# Autodesk Inventor assembly: Robot
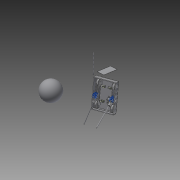
[picture p0: Inventor's stored thumbnail of the model, 180x180]
Saved by Autodesk Inventor 2014 (Build 180170000, 170)
## iProperties
Created: 2014-01-21
Part Number: Robot
Document SubType Name: Assembly
Designer: NilesStanton
Author: NilesStanton
## Documents named in this file (23)
- C:\GitHub\team3566-2014\CAD\Robot.iam
- C:\FIRST-2014-KOP\Additions\2014 Sidings.ipt
- C:\FIRST-2014-KOP\Motors\MOT_CIM-Motor_217-2000.iam
- C:\FIRST-2014-KOP\Additions\Flat Board.ipt
- C:\FIRST-2014-KOP\Additions\Front Paneling.ipt
- C:\FIRST-2014-KOP\Additions\3.5 in spacer.ipt
- C:\FIRST-2014-KOP\Additions\Mechanum Wheel.ipt
- C:\FIRST-2014-KOP\Additions\Gearbox.ipt
- C:\FIRST-2014-KOP\Additions\Long Bumber Wood.ipt
- C:\FIRST-2014-KOP\Additions\Short Bumper Wood.ipt
- C:\FIRST-2014-KOP\Drive Base Kit\DBK_TBMiniHousing-am-0650.ipt
- C:\FIRST-2014-KOP\Additions\El Tauro Horns.ipt
- C:\FIRST-2014-KOP\Additions\Tauro Vertical Pivot.ipt
- C:\FIRST-2014-KOP\Additions\Tauro Spacer.ipt
- C:\FIRST-2014-KOP\Additions\Tauro Vertical Pivot part 2.ipt
- C:\FIRST-2014-KOP\Additions\3.5 in pole.ipt
- C:\FIRST-2014-KOP\Additions\motor casing.ipt
- C:\FIRST-2014-KOP\Additions\.5 in spacer ring.ipt
- C:\FIRST-2014-KOP\Additions\winch triangle.ipt
- C:\FIRST-2014-KOP\Additions\Winch.ipt
- C:\FIRST-2014-KOP\Motors\MOT_GearMotor_am-0914.ipt
- C:\FIRST-2014-KOP\Additions\Bottom Board.ipt
- C:\GitHub\team3566-2014\CAD\ball.ipt
## Components (51 placed, 22 different names)
1. 2014 Sidings:1 — Flush:8, Mate:4, Angle:5, Flush:19, Flush:37, Flush:38, Flush:49, Mate:18
2. 2014 Sidings:2 — Mate:3, Flush:3, Angle:3, Flush:11, Flush:14, Flush:15, Tangent:7, Tangent:8, Flush:22, Flush:23, Flush:25, Flush:26, Flush:30, Flush:31, Mate:16
3. MOT_CIM-Motor_217-2000:1 [sub-assembly] — Tangent:9, Flush:30, Tangent:10
4. MOT_CIM-Motor_217-2000:2 [sub-assembly] — Flush:31, Tangent:11, Tangent:12
5. MOT_CIM-Motor_217-2000:3 [sub-assembly] — Flush:33, Tangent:15, Tangent:16
6. MOT_CIM-Motor_217-2000:4 [sub-assembly] — Flush:32, Tangent:13, Tangent:14
7. Flat Board:1
8. 2014 Sidings:3
9. Front Paneling:1 — Mate:2, Flush:2, Angle:2, Mate:3, Flush:3, Angle:3, Flush:24, Flush:27, Tangent:9, Tangent:15, Mate:7, Flush:55
10. Front Paneling:2 — Mate:1, Flush:1, Angle:1, Flush:5, Flush:7, Flush:9, Flush:10, Flush:18, Flush:21, Tangent:12, Tangent:13, Flush:36, Flush:39, Mate:6
11. 3.5 in spacer:1 — Flush:9, Flush:10, Flush:11, Flush:12, Flush:13, Mate:5, Angle:6, Tangent:1, Tangent:2
12. 3.5 in spacer:2 — Flush:5, Flush:6, Angle:4, Flush:7, Flush:8, Mate:4, Angle:5, Tangent:3, Tangent:4
13. 2014 Sidings:4 — Flush:12, Flush:13, Mate:5, Angle:6, Flush:34, Flush:35, Flush:52
14. 2014 Sidings:5 — Mate:1, Flush:1, Angle:1, Mate:2, Flush:2, Angle:2, Flush:6, Angle:4, Flush:16, Flush:17, Tangent:5, Tangent:6, Flush:20, Flush:28, Flush:29, Flush:32, Flush:33
15. Mechanum Wheel:1 — Flush:14, Tangent:1, Tangent:7
16. Mechanum Wheel:2 — Flush:17, Tangent:4, Tangent:5
17. Mechanum Wheel:3 — Flush:15, Tangent:2, Tangent:8
18. Mechanum Wheel:4 — Flush:16, Tangent:3, Tangent:6
19. Gearbox:1 — Flush:27, Flush:28, Flush:29, Tangent:16
20. Gearbox:2 — Flush:24, Flush:25, Flush:26, Tangent:10
21. Gearbox:3 — Flush:18, Flush:19, Flush:20, Tangent:14
22. Gearbox:4 — Flush:21, Flush:22, Flush:23, Tangent:11
23. Long Bumber Wood:1 — Flush:34, Flush:35, Flush:36, Flush:43, Flush:44, Flush:53
24. Long Bumber Wood:2 — Flush:37, Flush:38, Flush:39, Flush:41, Flush:42, Flush:50
25. Short Bumper Wood:1 — Flush:41, Mate:6, Flush:42, Tangent:21, Tangent:22
26. Short Bumper Wood:2 — Mate:7, Flush:43, Flush:44
27. DBK_TBMiniHousing-am-0650:1 — Insert:1, Flush:45, Flush:52, Flush:53
28. DBK_TBMiniHousing-am-0650:2 — Insert:2, Flush:45
29. El Tauro Horns:1
30. El Tauro Horns:2 — Mate:11, Insert:7
31. Tauro Vertical Pivot:1 — Insert:1, Insert:2, Insert:3, Tangent:22
32. Tauro Spacer:1 — Mate:8, Mate:9, Flush:46, Insert:3
33. Tauro Vertical Pivot part 2:1 — Mate:8, Mate:9, Flush:46, Insert:4, Insert:5
34. 3.5 in pole:1 — Insert:4, Insert:5, Insert:6
35. motor casing:1 — Insert:6, Mate:10, Tangent:17, Tangent:18
36. .5 in spacer ring:1 — Mate:10, Tangent:17, Tangent:18, Mate:11, Insert:7
37. DBK_TBMiniHousing-am-0650:3
38. DBK_TBMiniHousing-am-0650:4 — Flush:49, Flush:50
39. El Tauro Horns:3
40. Tauro Vertical Pivot:2 — Tangent:21
41. Tauro Spacer:2
42. Tauro Vertical Pivot part 2:2
43. 3.5 in pole:2
44. motor casing:2
45. .5 in spacer ring:2
46. winch triangle:1 — Insert:16, Flush:54
47. winch triangle:2 — Insert:15, Flush:54, Mate:17
48. Winch:1 — Insert:15, Insert:16, Insert:17
49. MOT_GearMotor_am-0914:1 — Insert:17, Mate:18
50. Bottom Board:1 — Mate:16, Flush:55, Mate:17
51. ball:1
## Relationships (115: Flush 52, Tangent 22, Mate 18, Insert 17, Angle 6)
- Mate:1: Front Paneling:2 ↔ 2014 Sidings:5
- Flush:1: Front Paneling:2 ↔ 2014 Sidings:5
- Angle:1 (90 deg): Front Paneling:2 ↔ 2014 Sidings:5
- Mate:2: Front Paneling:1 ↔ 2014 Sidings:5
- Flush:2: Front Paneling:1 ↔ 2014 Sidings:5
- Angle:2 (90 deg): Front Paneling:1 ↔ 2014 Sidings:5
- Mate:3: 2014 Sidings:2 ↔ Front Paneling:1
- Flush:3: 2014 Sidings:2 ↔ Front Paneling:1
- Angle:3 (90 deg): 2014 Sidings:2 ↔ Front Paneling:1
- Flush:5: Front Paneling:2 ↔ 3.5 in spacer:2
- Flush:6: 3.5 in spacer:2 ↔ 2014 Sidings:5
- Angle:4 (90 deg): 3.5 in spacer:2 ↔ 2014 Sidings:5
- Flush:7: Front Paneling:2 ↔ 3.5 in spacer:2
- Flush:8: 2014 Sidings:1 ↔ 3.5 in spacer:2
- Mate:4: 2014 Sidings:1 ↔ 3.5 in spacer:2
- Angle:5 (90 deg): 2014 Sidings:1 ↔ 3.5 in spacer:2
- Flush:9: Front Paneling:2 ↔ 3.5 in spacer:1
- Flush:10: Front Paneling:2 ↔ 3.5 in spacer:1
- Flush:11: 2014 Sidings:2 ↔ 3.5 in spacer:1
- Flush:12: 3.5 in spacer:1 ↔ 2014 Sidings:4
- Flush:13: 3.5 in spacer:1 ↔ 2014 Sidings:4
- Mate:5: 3.5 in spacer:1 ↔ 2014 Sidings:4
- Angle:6 (90 deg): 3.5 in spacer:1 ↔ 2014 Sidings:4
- Flush:14: 2014 Sidings:2 ↔ Mechanum Wheel:1
- Flush:15: 2014 Sidings:2 ↔ Mechanum Wheel:3
- Tangent:1 (50.8 mm): 3.5 in spacer:1 ↔ Mechanum Wheel:1
- Tangent:2 (622.3 mm): 3.5 in spacer:1 ↔ Mechanum Wheel:3
- Flush:16: 2014 Sidings:5 ↔ Mechanum Wheel:4
- Flush:17: 2014 Sidings:5 ↔ Mechanum Wheel:2
- Tangent:3 (50.8 mm): 3.5 in spacer:2 ↔ Mechanum Wheel:4
- Tangent:4 (622.3 mm): 3.5 in spacer:2 ↔ Mechanum Wheel:2
- Tangent:5 (-38.1 mm): 2014 Sidings:5 ↔ Mechanum Wheel:2
- Tangent:6 (-38.1 mm): 2014 Sidings:5 ↔ Mechanum Wheel:4
- Tangent:7 (-38.1 mm): 2014 Sidings:2 ↔ Mechanum Wheel:1
- Tangent:8 (-38.1 mm): 2014 Sidings:2 ↔ Mechanum Wheel:3
- Flush:18 (88.9 mm): Front Paneling:2 ↔ Gearbox:3
- Flush:19 (18.796 mm): 2014 Sidings:1 ↔ Gearbox:3
- Flush:20 (6.35 mm): 2014 Sidings:5 ↔ Gearbox:3
- Flush:21 (88.9 mm): Front Paneling:2 ↔ Gearbox:4
- Flush:22 (6.35 mm): 2014 Sidings:2 ↔ Gearbox:4
- Flush:23 (19.05 mm): 2014 Sidings:2 ↔ Gearbox:4
- Flush:24 (88.9 mm): Front Paneling:1 ↔ Gearbox:2
- Flush:25 (6.35 mm): 2014 Sidings:2 ↔ Gearbox:2
- Flush:26 (19.05 mm): 2014 Sidings:2 ↔ Gearbox:2
- Flush:27 (88.9 mm): Front Paneling:1 ↔ Gearbox:1
- Flush:28 (19.05 mm): 2014 Sidings:5 ↔ Gearbox:1
- Flush:29 (6.35 mm): 2014 Sidings:5 ↔ Gearbox:1
- Tangent:9 (215.9 mm): MOT_CIM-Motor_217-2000:1 ↔ Front Paneling:1
- Flush:30 (44.45 mm): 2014 Sidings:2 ↔ MOT_CIM-Motor_217-2000:1
- Tangent:10 (6.35 mm): MOT_CIM-Motor_217-2000:1 ↔ Gearbox:2
- Flush:31 (44.45 mm): 2014 Sidings:2 ↔ MOT_CIM-Motor_217-2000:2
- Tangent:11 (6.35 mm): MOT_CIM-Motor_217-2000:2 ↔ Gearbox:4
- Tangent:12 (215.9 mm): MOT_CIM-Motor_217-2000:2 ↔ Front Paneling:2
- Flush:32 (44.45 mm): MOT_CIM-Motor_217-2000:4 ↔ 2014 Sidings:5
- Tangent:13 (215.9 mm): MOT_CIM-Motor_217-2000:4 ↔ Front Paneling:2
- Tangent:14 (6.35 mm): MOT_CIM-Motor_217-2000:4 ↔ Gearbox:3
- Flush:33 (44.45 mm): MOT_CIM-Motor_217-2000:3 ↔ 2014 Sidings:5
- Tangent:15 (215.9 mm): MOT_CIM-Motor_217-2000:3 ↔ Front Paneling:1
- Tangent:16 (6.35 mm): MOT_CIM-Motor_217-2000:3 ↔ Gearbox:1
- Flush:34 (6.35 mm): 2014 Sidings:4 ↔ Long Bumber Wood:1
- Flush:35 (-76.2 mm): 2014 Sidings:4 ↔ Long Bumber Wood:1
- Flush:36: Front Paneling:2 ↔ Long Bumber Wood:1
- Flush:37 (6.35 mm): 2014 Sidings:1 ↔ Long Bumber Wood:2
- Flush:38 (-76.2 mm): 2014 Sidings:1 ↔ Long Bumber Wood:2
- Flush:39: Front Paneling:2 ↔ Long Bumber Wood:2
- Flush:41: Long Bumber Wood:2 ↔ Short Bumper Wood:1
- Mate:6: Front Paneling:2 ↔ Short Bumper Wood:1
- Flush:42: Long Bumber Wood:2 ↔ Short Bumper Wood:1
- Mate:7: Front Paneling:1 ↔ Short Bumper Wood:2
- Flush:43: Long Bumber Wood:1 ↔ Short Bumper Wood:2
- Flush:44: Long Bumber Wood:1 ↔ Short Bumper Wood:2
- Insert:1 (-50.8 mm): DBK_TBMiniHousing-am-0650:1 ↔ Tauro Vertical Pivot:1
- Insert:2 (-50.8 mm): DBK_TBMiniHousing-am-0650:2 ↔ Tauro Vertical Pivot:1
- Flush:45: DBK_TBMiniHousing-am-0650:1 ↔ DBK_TBMiniHousing-am-0650:2
- Mate:8: Tauro Spacer:1 ↔ Tauro Vertical Pivot part 2:1
- Mate:9 (19.05 mm): Tauro Spacer:1 ↔ Tauro Vertical Pivot part 2:1
- Flush:46 (3.175 mm): Tauro Spacer:1 ↔ Tauro Vertical Pivot part 2:1
- Insert:3 (-76.2 mm): Tauro Vertical Pivot:1 ↔ Tauro Spacer:1
- Insert:4: Tauro Vertical Pivot part 2:1 ↔ 3.5 in pole:1
- Insert:5: Tauro Vertical Pivot part 2:1 ↔ 3.5 in pole:1
- Insert:6 (6.35 mm): 3.5 in pole:1 ↔ motor casing:1
- Mate:10: motor casing:1 ↔ .5 in spacer ring:1
- Tangent:17 (38.1 mm): motor casing:1 ↔ .5 in spacer ring:1
- Tangent:18 (31.75 mm): motor casing:1 ↔ .5 in spacer ring:1
- Mate:11: El Tauro Horns:2 ↔ .5 in spacer ring:1
- Insert:7: El Tauro Horns:2 ↔ .5 in spacer ring:1
- [Insert] (-50.8 mm): DBK_TBMiniHousing-am-0650:3 ↔ Tauro Vertical Pivot:2
- [Insert] (-50.8 mm): DBK_TBMiniHousing-am-0650:4 ↔ Tauro Vertical Pivot:2
- [Flush]: DBK_TBMiniHousing-am-0650:3 ↔ DBK_TBMiniHousing-am-0650:4
- [Mate]: Tauro Spacer:2 ↔ Tauro Vertical Pivot part 2:2
- [Mate] (19.05 mm): Tauro Spacer:2 ↔ Tauro Vertical Pivot part 2:2
- [Flush] (3.175 mm): Tauro Spacer:2 ↔ Tauro Vertical Pivot part 2:2
- [Insert] (-76.2 mm): Tauro Vertical Pivot:2 ↔ Tauro Spacer:2
- [Insert]: Tauro Vertical Pivot part 2:2 ↔ 3.5 in pole:2
- [Insert]: Tauro Vertical Pivot part 2:2 ↔ 3.5 in pole:2
- [Insert] (6.35 mm): 3.5 in pole:2 ↔ motor casing:2
- [Mate]: motor casing:2 ↔ .5 in spacer ring:2
- [Tangent] (38.1 mm): motor casing:2 ↔ .5 in spacer ring:2
- [Tangent] (31.75 mm): motor casing:2 ↔ .5 in spacer ring:2
- [Mate]: El Tauro Horns:3 ↔ .5 in spacer ring:2
- [Insert]: El Tauro Horns:3 ↔ .5 in spacer ring:2
- Flush:49 (-25.4 mm): 2014 Sidings:1 ↔ DBK_TBMiniHousing-am-0650:4
- Flush:50 (45.72 mm): Long Bumber Wood:2 ↔ DBK_TBMiniHousing-am-0650:4
- Tangent:21 (342.9 mm): Short Bumper Wood:1 ↔ Tauro Vertical Pivot:2
- Flush:52 (-25.4 mm): 2014 Sidings:4 ↔ DBK_TBMiniHousing-am-0650:1
- Flush:53 (-45.72 mm): Long Bumber Wood:1 ↔ DBK_TBMiniHousing-am-0650:1
- Tangent:22 (-342.9 mm): Short Bumper Wood:1 ↔ Tauro Vertical Pivot:1
- Insert:15: winch triangle:2 ↔ Winch:1
- Insert:16: winch triangle:1 ↔ Winch:1
- Flush:54: winch triangle:1 ↔ winch triangle:2
- Insert:17 (-25.4 mm): Winch:1 ↔ MOT_GearMotor_am-0914:1
- Mate:16: 2014 Sidings:2 ↔ Bottom Board:1
- Flush:55: Front Paneling:1 ↔ Bottom Board:1
- Mate:17: winch triangle:2 ↔ Bottom Board:1
- Mate:18 (12.7 mm): 2014 Sidings:1 ↔ MOT_GearMotor_am-0914:1
## Named parameters: d160_d154 = 0 mm, d161_d155 = 38.1 mm, d162_d156 = 31.75 mm, d163_d157 = 0 mm, d164_d159 = 0 mm, d165_d149 = 6.35 mm, d166_d133 = -50.8 mm, d167_d135 = -50.8 mm, d168_d136 = 0 mm, d169_d140 = 0 mm, d170_d141 = 19.05 mm, d171_d142 = 3.175 mm, d172_d146 = -76.2 mm, d173_d147 = 0 mm, d174_d148 = 0 mm
